# Autodesk Inventor assembly: Moto
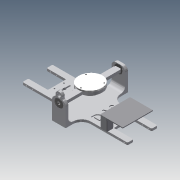
[picture p0: Inventor's stored thumbnail of the model, 180x180]
Saved by Autodesk Inventor 2019 (Build 230136000, 136)
## iProperties
Created: 2019-05-14
Part Number: Moto
Material: Genérico
Document SubType Name: Assembly
Designer: Daniel Regner
Mass: 72.4842 g
Surface Area: 627.234 cm^2
Volume: 112.761 cm^3
Density: 0.642811 g/cm^3
Author: Daniel Regner
## Documents named in this file (7)
- C:\Users\Daniel Regner\Documents\GitHub\Control-Gyro-stabilized-Motor\Mechanic\Inventor\Moto.iam
- C:\Users\Daniel Regner\Documents\GitHub\Control-Gyro-stabilized-Motor\Mechanic\Inventor\Chassis.ipt
- C:\Users\Daniel Regner\Documents\GitHub\Control-Gyro-stabilized-Motor\Mechanic\Inventor\Motor mount.ipt
- C:\Users\Daniel Regner\Documents\GitHub\Control-Gyro-stabilized-Motor\Mechanic\Inventor\electronics support.ipt
- C:\Users\Daniel Regner\Documents\GitHub\Control-Gyro-stabilized-Motor\Mechanic\Inventor\Moto\Design Accelerator\Rolamento1.iam
- C:\Users\Daniel Regner\Documents\GitHub\Control-Gyro-stabilized-Motor\Mechanic\Inventor\Moto\Design Accelerator\Rolamento2.iam
- C:\Users\Daniel Regner\Documents\GitHub\Control-Gyro-stabilized-Motor\Mechanic\Inventor\Motor mesh.ipt
## Components (6 placed, 5 different names)
1. Chassis:1 — Coincidência:1, Alinhamento:4, Coincidência:2, Coincidência:3, Coincidência:4, Coincidência:7, Coincidência:8, Coincidência:9, Coincidência:10, Alinhamento:5, Alinhamento:6, Coincidência:11
2. Motor mount:1 — Coincidência:1, Alinhamento:4, Coincidência:12, Coincidência:13
3. electronics support:1 — Coincidência:2, Coincidência:3, Coincidência:4
4. Rolamento:1 [sub-assembly] — Coincidência:9, Coincidência:10
5. Rolamento:2 [sub-assembly] — Coincidência:7, Coincidência:8
6. Motor mesh:1 — Coincidência:12, Coincidência:13
## Relationships (14: Mate 11, Flush 3)
- Coincidência:1 [Mate]: Chassis:1 ↔ Motor mount:1
- Alinhamento:4 [Flush]: Chassis:1 ↔ Motor mount:1
- Coincidência:2 [Mate]: Chassis:1 ↔ electronics support:1
- Coincidência:3 [Mate]: Chassis:1 ↔ electronics support:1
- Coincidência:4 [Mate]: Chassis:1 ↔ electronics support:1
- Coincidência:7 [Mate]: Chassis:1 ↔ Rolamento:2
- Coincidência:8 [Mate]: Chassis:1 ↔ Rolamento:2
- Coincidência:9 [Mate]: Chassis:1 ↔ Rolamento:1
- Coincidência:10 [Mate]: Chassis:1 ↔ Rolamento:1
- Alinhamento:5 [Flush]: Chassis:1
- Alinhamento:6 [Flush]: Chassis:1
- Coincidência:11 [Mate]: Chassis:1
- Coincidência:12 [Mate]: Motor mount:1 ↔ Motor mesh:1
- Coincidência:13 [Mate]: Motor mount:1 ↔ Motor mesh:1
